# Autodesk Inventor assembly: BatteryHousing
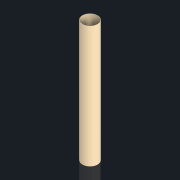
[picture p0: Inventor's stored thumbnail of the model, 180x180]
Saved by Autodesk Inventor 2022.2 (Build 262287000, 287)
## iProperties
Created: 2022-01-31
Part Number: BatteryHousing
Document SubType Name: Assembly
Designer: Michael Lacey
Mass: 80.7906 g
Surface Area: 366.818 cm^2
Volume: 82.4044 cm^3
Density: 0.980416 g/cm^3
Author: Michael Lacey
## Documents named in this file (3)
- C:\Users\foams\3D Objects\Light Saber\assembly test components\BatteryHousing.iam
- C:\Users\foams\3D Objects\Light Saber\assembly test components\InteralBatHousing.ipt
- C:\Users\foams\3D Objects\Light Saber\assembly test components\BigBattery.ipt
## Components (3 placed, 2 different names)
1. InteralBatHousing:1 — Mate:3
2. BigBattery:1 — Mate:4
3. BigBattery:3 — Mate:3, Mate:4
## Relationships (2: Mate 2)
- Mate:3: InteralBatHousing:1 ↔ BigBattery:3
- Mate:4: BigBattery:1 ↔ BigBattery:3
